# Autodesk Inventor assembly: NASA-20
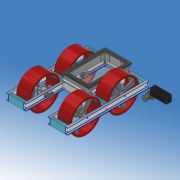
[picture p0: Inventor's stored thumbnail of the model, 180x180]
Saved by Autodesk Inventor 2020 (Build 240168000, 168)
## iProperties
RuleStatus: InUse
Created: 2019-09-05
Part Number: NASA-20
Document SubType Name: Assembly
Designer: Rick Szalay
Author: Rick Szalay
## Documents named in this file (24)
- C:\Users\mpark\Documents\NASA20\Inventor Files\NASA-20\NASA-20\NASA-20.iam
- C:\Users\mpark\Documents\NASA20\Inventor Files\NASA-20\NASA-20\A428.ipt
- C:\Users\mpark\Documents\NASA20\Inventor Files\NASA-20\NASA-20\NASA-20-WH-01.ipt
- C:\Users\mpark\Documents\NASA20\Inventor Files\NASA-20\NASA-20\NASA-20-WT-01.ipt
- C:\Users\mpark\Documents\NASA20\Inventor Files\NASA-20\NASA-20\FR\NASA-20-FR.iam
- C:\Users\mpark\Documents\NASA20\Inventor Files\NASA-20\NASA-20\FR\NASA-20-TB-01.ipt
- C:\Users\mpark\Documents\NASA20\Inventor Files\NASA-20\NASA-20\FR\NASA-20-OP-01.ipt
- C:\Users\mpark\Documents\NASA20\Inventor Files\NASA-20\NASA-20\FR\NASA-20-MP-01.ipt
- C:\Users\Matt\Documents\Inventor\Content Center Files\R2020\en-US\ANSI B18.2.1(3)\ANSI B18.2.1 - 1_4-20 UNC - 5.5(3).ipt
- C:\Users\Matt\Documents\Inventor\Content Center Files\R2020\en-US\ANSI B18.2.2(09)\ANSI B18.2.2 - 1_4 - 20(2).ipt
- C:\Users\mpark\Documents\NASA20\Inventor Files\NASA-20\NASA-20\Tube Replacements.iam
- C:\Users\mpark\Documents\NASA20\Inventor Files\NASA-20\NASA-20\E-Box\NASA-20-EBOX-B-01.ipt
- NASA-20-EBOX-B-01.ipt
- C:\Users\mpark\Documents\NASA20\Inventor Files\NASA-20\NASA-20\E-Box\NASA-20-EBOX-T-01.ipt
- NASA-20-EBOX-T-01.ipt
- C:\Users\mpark\Documents\NASA20\Inventor Files\NASA-20\NASA-20\E-Box\NASA-20-EBOX-T2-01.ipt
- C:\Users\mpark\Documents\NASA20\Inventor Files\NASA-20\NASA-20\E-Box\NASA-20-EBOX-LID-01.ipt
- C:\Users\mpark\Documents\NASA20\Inventor Files\NASA-20\NASA-20\E-Box\1603A230_UNFINISHED BRASS SURFACE-MNT HINGE W HOLES.ipt
- C:\Users\mpark\Documents\NASA20\Inventor Files\NASA-20\NASA-20\E-Box\9235K200_METAL 30 MM PANEL-MOUNT SWITCH.ipt
- C:\Users\mpark\Documents\NASA20\Inventor Files\NASA-20\NASA-20\E-Box\NASA-20-EBOX-EXT-01.iam
- C:\Users\mpark\Documents\NASA20\Inventor Files\NASA-20\NASA-20\E-Box\NASA-20-EBOX-LID-REV1-01.ipt
- C:\Users\mpark\Documents\NASA20\Inventor Files\NASA-20\NASA-20\E-Box\NASA-20-EBOX-LID-HANDLE-01.ipt
- C:\Users\mpark\OneDrive\Documents\Inventor\Content Center Files\R2020\en-US\AS 1420\AS 1420 - 1973 - M5 x 20.ipt
- C:\Users\mpark\Documents\NASA20\Inventor Files\NASA-20\MaxAmps_battery.ipt
## Components (92 placed, 21 different names)
1. A428:1 — Mate:38, Mate:39, Flush:28, Mate:41
2. NASA-20-WH-01:1 — Mate:6, Flush:9, Mate:40, Mate:41
3. NASA-20-WT-01:1 — Mate:6, Flush:9, Mate:61, Tangent:1
4. NASA-20-FR:1 [sub-assembly] — Mate:20, Mate:21, Flush:13, Mate:22, Mate:23, Mate:24, Mate:25, Mate:26, Mate:27, Mate:28, Mate:29, Mate:30, Mate:31, Mate:32, Mate:33, Mate:34, Mate:35, Flush:26, Flush:27, Flush:29, Mate:42, Mate:58, Flush:36, Mate:59, Mate:60, Flush:37, Flush:38, Insert:13, Insert:14, Insert:15, Insert:16, Insert:17, Insert:18, Insert:19, Insert:20, Insert:21, Insert:22, Insert:23, Insert:24, Mate:64, Mate:65, Mate:66, Mate:67, Mate:68, Mate:69, Mate:70, Mate:71, Mate:72, Mate:73, Mate:74, Mate:75, Mate:76, Mate:77, Mate:78, Mate:79, Mate:80, Mate:81, Mate:82, Mate:83, Flush:39, Flush:40, Flush:41, Flush:42, Flush:51, Flush:53, Flush:54, Mate:120
5. NASA-20-OP-01:1 — Flush:24, Flush:25, Mate:37, Flush:26, Flush:27, Mate:63, Insert:7, Insert:8, Insert:9, Insert:10, Insert:11, Insert:12
6. NASA-20-OP-01:2 — Flush:24, Flush:25, Mate:36, Insert:1, Insert:2, Insert:3, Insert:4, Insert:5, Insert:6
7. NASA-20-MP-01:1 — Mate:38, Mate:39, Flush:28, Mate:40, Flush:29, Mate:42
8. A428:2
9. NASA-20-WH-01:2
10. NASA-20-WT-01:2 — Mate:62, Tangent:1
11. NASA-20-MP-01:2 — Mate:58, Flush:36
12. A428:3
13. NASA-20-WH-01:3
14. NASA-20-WT-01:3 — Mate:62, Mate:63
15. NASA-20-MP-01:3 — Mate:59, Flush:37
16. A428:4
17. NASA-20-WH-01:4
18. NASA-20-WT-01:4 — Mate:61
19. NASA-20-MP-01:4 — Mate:60, Flush:38
20. NASA-20-EBOX-LID-HANDLE-01:1 — Mate:123, Flush:58, Flush:59
21. MaxAmps_battery:1
22. 9235K200_METAL 30 MM PANEL-MOUNT SWITCH:2
23. NASA-20-TB-01:1 — Flush:14, Mate:22, Mate:23
24. NASA-20-TB-01:2 — Flush:14, Flush:15, Mate:24, Mate:36
25. NASA-20-TB-01:3 — Flush:15, Flush:16, Mate:25
26. NASA-20-TB-01:4 — Flush:16, Flush:17, Mate:26
27. NASA-20-TB-01:5 — Flush:17, Flush:18, Mate:27
28. NASA-20-TB-01:6 — Flush:18, Mate:28
29. NASA-20-TB-01:7 — Mate:34, Mate:37
30. NASA-20-TB-01:8 — Mate:35
31. NASA-20-TB-01:9 — Mate:30
32. NASA-20-TB-01:10 — Mate:33
33. NASA-20-TB-01:11 — Mate:32
34. NASA-20-TB-01:12 — Mate:29, Mate:31
35. AS 1420 - Metric M5 x 20:11 — Insert:39
36. AS 1420 - Metric M5 x 20:12 — Insert:40
37. AS 1420 - Metric M5 x 20:13 — Insert:41
38. AS 1420 - Metric M5 x 20:14 — Insert:42
39. AS 1420 - Metric M5 x 20:15 — Insert:43
40. AS 1420 - Metric M5 x 20:16 — Insert:44
41. AS 1420 - Metric M5 x 20:1 — Insert:45
42. AS 1420 - Metric M5 x 20:17 — Insert:46
43. AS 1420 - Metric M5 x 20:18 — Insert:47
44. AS 1420 - Metric M5 x 20:19 — Insert:48
45. AS 1420 - Metric M5 x 20:2 — Insert:29
46. AS 1420 - Metric M5 x 20:3 — Insert:30
47. AS 1420 - Metric M5 x 20:4 — Insert:32
48. AS 1420 - Metric M5 x 20:5 — Insert:33
49. AS 1420 - Metric M5 x 20:6 — Insert:34
50. AS 1420 - Metric M5 x 20:7 — Insert:35
51. AS 1420 - Metric M5 x 20:8 — Insert:36
52. AS 1420 - Metric M5 x 20:9 — Insert:37
53. AS 1420 - Metric M5 x 20:10 — Insert:38
54. Hex Cap Screw - Inch 1/4-20 UNC - 5.5:13 — Insert:1
55. Hex Cap Screw - Inch 1/4-20 UNC - 5.5:14 — Insert:2
56. Hex Cap Screw - Inch 1/4-20 UNC - 5.5:15 — Insert:3
57. Hex Cap Screw - Inch 1/4-20 UNC - 5.5:16 — Insert:4
58. Hex Cap Screw - Inch 1/4-20 UNC - 5.5:17 — Insert:5
59. Hex Cap Screw - Inch 1/4-20 UNC - 5.5:18 — Insert:6
60. Hex Cap Screw - Inch 1/4-20 UNC - 5.5:20 — Insert:7
61. Hex Cap Screw - Inch 1/4-20 UNC - 5.5:19 — Insert:8
62. Hex Cap Screw - Inch 1/4-20 UNC - 5.5:21 — Insert:9
63. Hex Cap Screw - Inch 1/4-20 UNC - 5.5:22 — Insert:10
64. Hex Cap Screw - Inch 1/4-20 UNC - 5.5:23 — Insert:11
65. Hex Cap Screw - Inch 1/4-20 UNC - 5.5:24 — Insert:12
66. Hex Nut - Inch 1/4 - 20:13 — Insert:13
67. Hex Nut - Inch 1/4 - 20:14 — Insert:14
68. Hex Nut - Inch 1/4 - 20:15 — Insert:15
69. Hex Nut - Inch 1/4 - 20:16 — Insert:16
70. Hex Nut - Inch 1/4 - 20:17 — Insert:17
71. Hex Nut - Inch 1/4 - 20:18 — Insert:18
72. Hex Nut - Inch 1/4 - 20:19 — Insert:19
73. Hex Nut - Inch 1/4 - 20:20 — Insert:20
74. Hex Nut - Inch 1/4 - 20:21 — Insert:21
75. Hex Nut - Inch 1/4 - 20:22 — Insert:22
76. Hex Nut - Inch 1/4 - 20:23 — Insert:23
77. Hex Nut - Inch 1/4 - 20:24 — Insert:24
78. Tube Replacements:1 [sub-assembly] — Mate:64, Mate:70, Mate:81
79. Tube Replacements:2 [sub-assembly] — Mate:65, Mate:72, Mate:80
80. Tube Replacements:3 [sub-assembly] — Mate:66, Mate:71, Mate:79
81. Tube Replacements:4 [sub-assembly] — Mate:69, Mate:75, Mate:76
82. Tube Replacements:5 [sub-assembly] — Mate:68, Mate:74, Mate:77
83. Tube Replacements:6 [sub-assembly] — Mate:67, Mate:73, Mate:78
84. 9235K200_METAL 30 MM PANEL-MOUNT SWITCH:1
85. 1603A230_UNFINISHED BRASS SURFACE-MNT HINGE W HOLES:1 — Mate:90, Flush:49, Flush:50, Flush:51
86. 1603A230_UNFINISHED BRASS SURFACE-MNT HINGE W HOLES:2 — Mate:91, Flush:48, Flush:50
87. NASA-20-EBOX-LID-01:1 — Mate:85, Flush:45, Mate:86, Mate:87
88. NASA-20-EBOX-T2-01:2 — Mate:84, Flush:43, Flush:44, Flush:45, Mate:86, Mate:87, Mate:90, Mate:91, Flush:48, Flush:49, Insert:29, Insert:30, Insert:32, Insert:33, Insert:34, Insert:35, Insert:36, Insert:37, Insert:38
89. NASA-20-EBOX-T-01:1 — Mate:83, Flush:41, Flush:42, Mate:84, Flush:43, Flush:44, Mate:85
90. NASA-20-EBOX-B-01:1 — Mate:82, Flush:39, Flush:40, Insert:39, Insert:40, Insert:41, Insert:42, Insert:43, Insert:44, Insert:45, Insert:46, Insert:47, Insert:48
91. NASA-20-EBOX-EXT-01:1 [sub-assembly] — Flush:53, Flush:54, Mate:120, Mate:122, Flush:56, Flush:57, Flush:58, Flush:59
92. NASA-20-EBOX-LID-REV1-01:1 — Mate:122, Flush:56, Flush:57, Mate:123
## Relationships (162: Mate 74, Flush 44, Insert 43, Tangent 1)
- Mate:6: NASA-20-WH-01:1 ↔ NASA-20-WT-01:1
- Flush:9 (19.05 mm): NASA-20-WH-01:1 ↔ NASA-20-WT-01:1
- Mate:20: NASA-20-FR:1
- Mate:21: NASA-20-FR:1
- Flush:13: NASA-20-FR:1
- Flush:14: NASA-20-TB-01:1 ↔ NASA-20-TB-01:2
- Flush:15: NASA-20-TB-01:2 ↔ NASA-20-TB-01:3
- Flush:16: NASA-20-TB-01:3 ↔ NASA-20-TB-01:4
- Flush:17: NASA-20-TB-01:4 ↔ NASA-20-TB-01:5
- Flush:18: NASA-20-TB-01:5 ↔ NASA-20-TB-01:6
- Mate:22: NASA-20-FR:1 ↔ NASA-20-TB-01:1
- Mate:23: NASA-20-FR:1 ↔ NASA-20-TB-01:1
- Mate:24: NASA-20-FR:1 ↔ NASA-20-TB-01:2
- Mate:25: NASA-20-FR:1 ↔ NASA-20-TB-01:3
- Mate:26: NASA-20-FR:1 ↔ NASA-20-TB-01:4
- Mate:27: NASA-20-FR:1 ↔ NASA-20-TB-01:5
- Mate:28: NASA-20-FR:1 ↔ NASA-20-TB-01:6
- [Flush]: NASA-20-TB-01:7 ↔ NASA-20-TB-01:8
- [Flush]: NASA-20-TB-01:8 ↔ NASA-20-TB-01:9
- [Flush]: NASA-20-TB-01:9 ↔ NASA-20-TB-01:10
- [Flush]: NASA-20-TB-01:10 ↔ NASA-20-TB-01:11
- [Flush]: NASA-20-TB-01:11 ↔ NASA-20-TB-01:12
- Mate:29: NASA-20-FR:1 ↔ NASA-20-TB-01:12
- Mate:30: NASA-20-FR:1 ↔ NASA-20-TB-01:9
- Mate:31: NASA-20-FR:1 ↔ NASA-20-TB-01:12
- Mate:32: NASA-20-FR:1 ↔ NASA-20-TB-01:11
- Mate:33: NASA-20-FR:1 ↔ NASA-20-TB-01:10
- Mate:34: NASA-20-FR:1 ↔ NASA-20-TB-01:7
- Mate:35: NASA-20-FR:1 ↔ NASA-20-TB-01:8
- Flush:24: NASA-20-OP-01:1 ↔ NASA-20-OP-01:2
- Flush:25: NASA-20-OP-01:1 ↔ NASA-20-OP-01:2
- Mate:36: NASA-20-OP-01:2 ↔ NASA-20-TB-01:2
- Mate:37: NASA-20-OP-01:1 ↔ NASA-20-TB-01:7
- Flush:26: NASA-20-FR:1 ↔ NASA-20-OP-01:1
- Flush:27: NASA-20-FR:1 ↔ NASA-20-OP-01:1
- Mate:38: A428:1 ↔ NASA-20-MP-01:1
- Mate:39: A428:1 ↔ NASA-20-MP-01:1
- Flush:28: A428:1 ↔ NASA-20-MP-01:1
- Mate:40 (1.5875 mm): NASA-20-WH-01:1 ↔ NASA-20-MP-01:1
- Mate:41: A428:1 ↔ NASA-20-WH-01:1
- Flush:29: NASA-20-FR:1 ↔ NASA-20-MP-01:1
- Mate:42: NASA-20-FR:1 ↔ NASA-20-MP-01:1
- [Mate]: NASA-20-WH-01:2 ↔ NASA-20-WT-01:2
- [Flush] (19.05 mm): NASA-20-WH-01:2 ↔ NASA-20-WT-01:2
- [Mate]: A428:2 ↔ NASA-20-MP-01:2
- [Mate]: A428:2 ↔ NASA-20-MP-01:2
- [Flush]: A428:2 ↔ NASA-20-MP-01:2
- [Mate] (1.5875 mm): NASA-20-WH-01:2 ↔ NASA-20-MP-01:2
- [Mate]: A428:2 ↔ NASA-20-WH-01:2
- [Mate]: NASA-20-WH-01:3 ↔ NASA-20-WT-01:3
- [Flush] (19.05 mm): NASA-20-WH-01:3 ↔ NASA-20-WT-01:3
- [Mate]: A428:3 ↔ NASA-20-MP-01:3
- [Mate]: A428:3 ↔ NASA-20-MP-01:3
- [Flush]: A428:3 ↔ NASA-20-MP-01:3
- [Mate] (1.5875 mm): NASA-20-WH-01:3 ↔ NASA-20-MP-01:3
- [Mate]: A428:3 ↔ NASA-20-WH-01:3
- [Mate]: NASA-20-WH-01:4 ↔ NASA-20-WT-01:4
- [Flush] (19.05 mm): NASA-20-WH-01:4 ↔ NASA-20-WT-01:4
- [Mate]: A428:4 ↔ NASA-20-MP-01:4
- [Mate]: A428:4 ↔ NASA-20-MP-01:4
- [Flush]: A428:4 ↔ NASA-20-MP-01:4
- [Mate] (1.5875 mm): NASA-20-WH-01:4 ↔ NASA-20-MP-01:4
- [Mate]: A428:4 ↔ NASA-20-WH-01:4
- Mate:58: NASA-20-FR:1 ↔ NASA-20-MP-01:2
- Flush:36: NASA-20-FR:1 ↔ NASA-20-MP-01:2
- Mate:59: NASA-20-FR:1 ↔ NASA-20-MP-01:3
- Mate:60: NASA-20-FR:1 ↔ NASA-20-MP-01:4
- Flush:37: NASA-20-FR:1 ↔ NASA-20-MP-01:3
- Flush:38: NASA-20-FR:1 ↔ NASA-20-MP-01:4
- Mate:61: NASA-20-WT-01:1 ↔ NASA-20-WT-01:4
- Mate:62: NASA-20-WT-01:2 ↔ NASA-20-WT-01:3
- Tangent:1 (50.8 mm): NASA-20-WT-01:1 ↔ NASA-20-WT-01:2
- Mate:63: NASA-20-OP-01:1 ↔ NASA-20-WT-01:3
- Insert:1: NASA-20-OP-01:2 ↔ Hex Cap Screw - Inch 1/4-20 UNC - 5.5:13
- Insert:2: NASA-20-OP-01:2 ↔ Hex Cap Screw - Inch 1/4-20 UNC - 5.5:14
- Insert:3: NASA-20-OP-01:2 ↔ Hex Cap Screw - Inch 1/4-20 UNC - 5.5:15
- Insert:4: NASA-20-OP-01:2 ↔ Hex Cap Screw - Inch 1/4-20 UNC - 5.5:16
- Insert:5: NASA-20-OP-01:2 ↔ Hex Cap Screw - Inch 1/4-20 UNC - 5.5:17
- Insert:6: NASA-20-OP-01:2 ↔ Hex Cap Screw - Inch 1/4-20 UNC - 5.5:18
- Insert:7: NASA-20-OP-01:1 ↔ Hex Cap Screw - Inch 1/4-20 UNC - 5.5:20
- Insert:8: NASA-20-OP-01:1 ↔ Hex Cap Screw - Inch 1/4-20 UNC - 5.5:19
- Insert:9: NASA-20-OP-01:1 ↔ Hex Cap Screw - Inch 1/4-20 UNC - 5.5:21
- Insert:10: NASA-20-OP-01:1 ↔ Hex Cap Screw - Inch 1/4-20 UNC - 5.5:22
- Insert:11: NASA-20-OP-01:1 ↔ Hex Cap Screw - Inch 1/4-20 UNC - 5.5:23
- Insert:12: NASA-20-OP-01:1 ↔ Hex Cap Screw - Inch 1/4-20 UNC - 5.5:24
- Insert:13: NASA-20-FR:1 ↔ Hex Nut - Inch 1/4 - 20:13
- Insert:14: NASA-20-FR:1 ↔ Hex Nut - Inch 1/4 - 20:14
- Insert:15: NASA-20-FR:1 ↔ Hex Nut - Inch 1/4 - 20:15
- Insert:16: NASA-20-FR:1 ↔ Hex Nut - Inch 1/4 - 20:16
- Insert:17: NASA-20-FR:1 ↔ Hex Nut - Inch 1/4 - 20:17
- Insert:18: NASA-20-FR:1 ↔ Hex Nut - Inch 1/4 - 20:18
- Insert:19: NASA-20-FR:1 ↔ Hex Nut - Inch 1/4 - 20:19
- Insert:20: NASA-20-FR:1 ↔ Hex Nut - Inch 1/4 - 20:20
- Insert:21: NASA-20-FR:1 ↔ Hex Nut - Inch 1/4 - 20:21
- Insert:22: NASA-20-FR:1 ↔ Hex Nut - Inch 1/4 - 20:22
- Insert:23: NASA-20-FR:1 ↔ Hex Nut - Inch 1/4 - 20:23
- Insert:24: NASA-20-FR:1 ↔ Hex Nut - Inch 1/4 - 20:24
- Mate:64: NASA-20-FR:1 ↔ Tube Replacements:1
- Mate:65: NASA-20-FR:1 ↔ Tube Replacements:2
- Mate:66: NASA-20-FR:1 ↔ Tube Replacements:3
- Mate:67: NASA-20-FR:1 ↔ Tube Replacements:6
- Mate:68: NASA-20-FR:1 ↔ Tube Replacements:5
- Mate:69: NASA-20-FR:1 ↔ Tube Replacements:4
- Mate:70: NASA-20-FR:1 ↔ Tube Replacements:1
- Mate:71: NASA-20-FR:1 ↔ Tube Replacements:3
- Mate:72: NASA-20-FR:1 ↔ Tube Replacements:2
- Mate:73: NASA-20-FR:1 ↔ Tube Replacements:6
- Mate:74: NASA-20-FR:1 ↔ Tube Replacements:5
- Mate:75: NASA-20-FR:1 ↔ Tube Replacements:4
- Mate:76: NASA-20-FR:1 ↔ Tube Replacements:4
- Mate:77: NASA-20-FR:1 ↔ Tube Replacements:5
- Mate:78: NASA-20-FR:1 ↔ Tube Replacements:6
- Mate:79: NASA-20-FR:1 ↔ Tube Replacements:3
- Mate:80: NASA-20-FR:1 ↔ Tube Replacements:2
- Mate:81: NASA-20-FR:1 ↔ Tube Replacements:1
- Mate:82: NASA-20-FR:1 ↔ NASA-20-EBOX-B-01:1
- Mate:83: NASA-20-FR:1 ↔ NASA-20-EBOX-T-01:1
- Flush:39: NASA-20-FR:1 ↔ NASA-20-EBOX-B-01:1
- Flush:40: NASA-20-FR:1 ↔ NASA-20-EBOX-B-01:1
- Flush:41: NASA-20-FR:1 ↔ NASA-20-EBOX-T-01:1
- Flush:42: NASA-20-FR:1 ↔ NASA-20-EBOX-T-01:1
- Mate:84: NASA-20-EBOX-T2-01:2 ↔ NASA-20-EBOX-T-01:1
- Flush:43: NASA-20-EBOX-T2-01:2 ↔ NASA-20-EBOX-T-01:1
- Flush:44: NASA-20-EBOX-T2-01:2 ↔ NASA-20-EBOX-T-01:1
- Mate:85: NASA-20-EBOX-LID-01:1 ↔ NASA-20-EBOX-T-01:1
- Flush:45: NASA-20-EBOX-LID-01:1 ↔ NASA-20-EBOX-T2-01:2
- Mate:86 (1 mm): NASA-20-EBOX-LID-01:1 ↔ NASA-20-EBOX-T2-01:2
- Mate:87 (1 mm): NASA-20-EBOX-LID-01:1 ↔ NASA-20-EBOX-T2-01:2
- Mate:90: 1603A230_UNFINISHED BRASS SURFACE-MNT HINGE W HOLES:1 ↔ NASA-20-EBOX-T2-01:2
- Mate:91: 1603A230_UNFINISHED BRASS SURFACE-MNT HINGE W HOLES:2 ↔ NASA-20-EBOX-T2-01:2
- Flush:48 (38.1 mm): 1603A230_UNFINISHED BRASS SURFACE-MNT HINGE W HOLES:2 ↔ NASA-20-EBOX-T2-01:2
- Flush:49 (38.1 mm): 1603A230_UNFINISHED BRASS SURFACE-MNT HINGE W HOLES:1 ↔ NASA-20-EBOX-T2-01:2
- Flush:50: 1603A230_UNFINISHED BRASS SURFACE-MNT HINGE W HOLES:1 ↔ 1603A230_UNFINISHED BRASS SURFACE-MNT HINGE W HOLES:2
- Flush:51 (25.4 mm): NASA-20-FR:1 ↔ 1603A230_UNFINISHED BRASS SURFACE-MNT HINGE W HOLES:1
- Insert:29: AS 1420 - Metric M5 x 20:2 ↔ NASA-20-EBOX-T2-01:2
- Insert:30: AS 1420 - Metric M5 x 20:3 ↔ NASA-20-EBOX-T2-01:2
- Insert:32: AS 1420 - Metric M5 x 20:4 ↔ NASA-20-EBOX-T2-01:2
- Insert:33: AS 1420 - Metric M5 x 20:5 ↔ NASA-20-EBOX-T2-01:2
- Insert:34: AS 1420 - Metric M5 x 20:6 ↔ NASA-20-EBOX-T2-01:2
- Insert:35: AS 1420 - Metric M5 x 20:7 ↔ NASA-20-EBOX-T2-01:2
- Insert:36: AS 1420 - Metric M5 x 20:8 ↔ NASA-20-EBOX-T2-01:2
- Insert:37: AS 1420 - Metric M5 x 20:9 ↔ NASA-20-EBOX-T2-01:2
- Insert:38: AS 1420 - Metric M5 x 20:10 ↔ NASA-20-EBOX-T2-01:2
- Insert:39: AS 1420 - Metric M5 x 20:11 ↔ NASA-20-EBOX-B-01:1
- Insert:40: AS 1420 - Metric M5 x 20:12 ↔ NASA-20-EBOX-B-01:1
- Insert:41: AS 1420 - Metric M5 x 20:13 ↔ NASA-20-EBOX-B-01:1
- Insert:42: AS 1420 - Metric M5 x 20:14 ↔ NASA-20-EBOX-B-01:1
- Insert:43: AS 1420 - Metric M5 x 20:15 ↔ NASA-20-EBOX-B-01:1
- Insert:44: AS 1420 - Metric M5 x 20:16 ↔ NASA-20-EBOX-B-01:1
- Insert:45: AS 1420 - Metric M5 x 20:1 ↔ NASA-20-EBOX-B-01:1
- Insert:46: AS 1420 - Metric M5 x 20:17 ↔ NASA-20-EBOX-B-01:1
- Insert:47: AS 1420 - Metric M5 x 20:18 ↔ NASA-20-EBOX-B-01:1
- Insert:48: AS 1420 - Metric M5 x 20:19 ↔ NASA-20-EBOX-B-01:1
- Flush:53: NASA-20-FR:1 ↔ NASA-20-EBOX-EXT-01:1
- Flush:54: NASA-20-FR:1 ↔ NASA-20-EBOX-EXT-01:1
- Mate:120: NASA-20-FR:1 ↔ NASA-20-EBOX-EXT-01:1
- Mate:122: NASA-20-EBOX-EXT-01:1 ↔ NASA-20-EBOX-LID-REV1-01:1
- Flush:56: NASA-20-EBOX-EXT-01:1 ↔ NASA-20-EBOX-LID-REV1-01:1
- Flush:57: NASA-20-EBOX-EXT-01:1 ↔ NASA-20-EBOX-LID-REV1-01:1
- Mate:123: NASA-20-EBOX-LID-HANDLE-01:1 ↔ NASA-20-EBOX-LID-REV1-01:1
- Flush:58 (-31.75 mm): NASA-20-EBOX-LID-HANDLE-01:1 ↔ NASA-20-EBOX-EXT-01:1
- Flush:59 (76.2 mm): NASA-20-EBOX-LID-HANDLE-01:1 ↔ NASA-20-EBOX-EXT-01:1
## Named parameters: d53_d41 = 0 mm, d54_d42 = 0 mm, d55_d43 = 0 mm, d56_d44 = 0 mm, d57_d45 = 0 mm, d78_d71 = 0 mm, d79_d72 = 0 mm, d80_d73 = 0 mm, d81_d74 = 1.5875 mm, d82_d75 = 0 mm, d83_d14 = 0 mm, d84_d15 = 19.05 mm, d85_d71 = 0 mm, d86_d72 = 0 mm, d87_d73 = 0 mm, d88_d74 = 1.5875 mm, d89_d75 = 0 mm, d90_d14 = 0 mm, d91_d15 = 19.05 mm, d92_d71 = 0 mm, d93_d72 = 0 mm, d94_d73 = 0 mm, d95_d74 = 1.5875 mm, d96_d75 = 0 mm, d97_d14 = 0 mm, d98_d15 = 19.05 mm
